# Autodesk Inventor assembly: fox
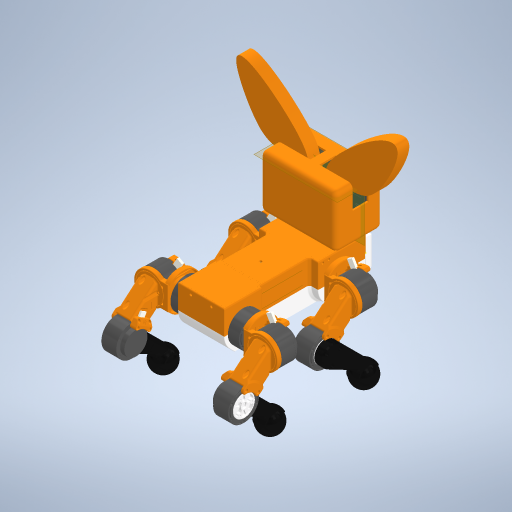
[picture p0: Inventor's stored thumbnail of the model, 512x512]
Saved by Autodesk Inventor 2024.2 (Build 282272000, 272)
## iProperties
Created: 2025-09-19
Part Number: fox
Document SubType Name: Assembly
Designer: AdminForWorker
Title: Pupper v3.5 v16
Author: AdminForWorker
## Documents named in this file (10)
- D:\dog\construction\fox\fox.iam
- D:\dog\construction\fox\legs\Lower leg - Short Short V6 (No Pinch) v20.iam
- D:\dog\construction\fox\legs\Lower leg - Short Short V6 (No Pinch) v20_1.iam
- D:\dog\construction\fox\legs\две части ног.iam
- D:\dog\construction\fox\body\тело лисы.iam
- D:\dog\construction\fox\legs\одна часть ноги.iam
- D:\dog\construction\fox\legs\одна часть ноги симетр.iam
- D:\dog\construction\fox\legs\Lower leg - Short Short V6 (No Pinch) v20(Mirror).iam
- D:\dog\construction\fox\legs\Lower leg - Short Short V6 (No Pinch) v20(Mirror)_1.iam
- D:\dog\construction\fox\body\аккумулятор 21700.iam
## Components (9 placed, 9 different names)
1. нижняя нога правая 2 [sub-assembly]
2. тело [sub-assembly] — Совмещение:1, Совмещение:2, Заподлицо:1
3. верхняя нога левая [sub-assembly] — Совмещение:3
4. верхняя нога правая [sub-assembly]
5. нижняя нога левая 2 [sub-assembly] — Совмещение:3
6. нижняя нога левая [sub-assembly]
7. нижняя нога правая [sub-assembly]
8. верхняя нога перед [sub-assembly]
9. аккумулятор 21700:1 [sub-assembly] — Совмещение:1, Совмещение:2, Заподлицо:1
## Relationships (4: Mate 3, Flush 1)
- Совмещение:1 [Mate] (4 mm): тело ↔ аккумулятор 21700:1
- Совмещение:2 [Mate] (11 mm): тело ↔ аккумулятор 21700:1
- Заподлицо:1 [Flush]: тело ↔ аккумулятор 21700:1
- Совмещение:3 [Mate]: верхняя нога левая ↔ нижняя нога левая 2
